# Autodesk Inventor assembly: MotorSide
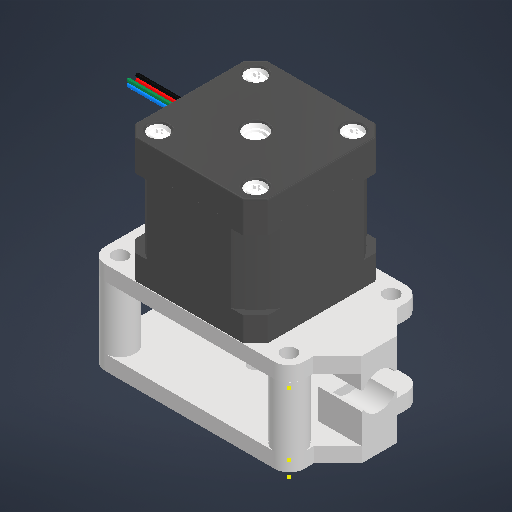
[picture p0: Inventor's stored thumbnail of the model, 512x512]
Saved by Autodesk Inventor 2026 (Build 300175000, 175)
## iProperties
Created: 2025-04-11
Part Number: MotorSide
Document SubType Name: Assembly
Designer: jjgen
Author: jjgen
## Documents named in this file (4)
- C:\Users\jjgen\OneDrive\Documents\Inventor\Curtain Opener\MotorSide.iam
- C:\Users\jjgen\OneDrive\Documents\Inventor\Curtain Opener\MotorBot.ipt
- C:\Users\jjgen\OneDrive\Documents\Inventor\Curtain Opener\MotorTop.ipt
- C:\Users\jjgen\OneDrive\Documents\Inventor\Curtain Opener\17HS16-2004S1.ipt
## Components (3 placed, 3 different names)
1. MotorBot:1 — Mate:1, Mate:2
2. MotorTop:1 — Mate:1, Mate:2, Mate:3
3. 17HS16-2004S1:1 — Mate:3
## Relationships (3: Mate 3)
- Mate:1: MotorBot:1 ↔ MotorTop:1
- Mate:2: MotorBot:1 ↔ MotorTop:1
- Mate:3: MotorTop:1 ↔ 17HS16-2004S1:1
